# Autodesk Inventor assembly: Schlitten
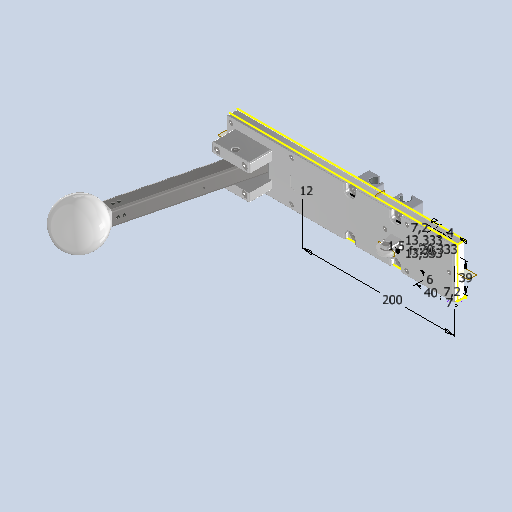
[picture p0: Inventor's stored thumbnail of the model, 512x512]
Saved by Autodesk Inventor 2025 (Build 290162010, 162A)
## iProperties
Created: 2024-11-25
Part Number: Schlitten
Document SubType Name: Assembly
Designer: Admin
Mass: 1140.3 g
Surface Area: 1828.97 cm^2
Volume: 452.563 cm^3
Density: 2.51965 g/cm^3
Author: Admin
## Documents named in this file (21)
- C:\Users\Admin\GIT\HDVKBM\CAD\Krandemonstrator\Schlitten.iam
- C:\Users\Admin\Documents\Inventor\Content Center Files\R2025\de-DE\BS 1804\BS 1804-2 - 2 x 10.ipt
- C:\Users\Admin\GIT\HDVKBM\CAD\Krandemonstrator\SchlittenS.ipt
- C:\Users\Admin\GIT\HDVKBM\CAD\Krandemonstrator\WJ200UM_01_10_1\WJ200UM_01_10_1.iam
- C:\Users\Admin\Documents\Inventor\Content Center Files\R2025\de-DE\DIN 7991(2)\DIN 7991 - M6x16.ipt
- C:\Users\Admin\GIT\HDVKBM\CAD\Krandemonstrator\SchlittenDeckel.ipt
- C:\Users\Admin\Documents\Inventor\Content Center Files\R2025\de-DE\AS 1427(03)\AS 1427 - M2 x 10(1).ipt
- C:\Users\Admin\GIT\HDVKBM\CAD\Krandemonstrator\UmlenkrolleHalterHeavy.iam
- C:\Users\Admin\GIT\HDVKBM\CAD\Krandemonstrator\Bedienhebel.iam
- C:\Users\Admin\GIT\HDVKBM\CAD\Krandemonstrator\SeilspannerDraht.ipt
- C:\Users\Admin\Documents\Inventor\Content Center Files\R2025\de-DE\DIN 7991(2)\DIN 7991 - M3x10.ipt
- C:\Users\Admin\GIT\HDVKBM\CAD\Krandemonstrator\SchlittenDeckelHinten.ipt
- C:\Users\Admin\GIT\HDVKBM\CAD\Krandemonstrator\SchlittenDeckelMitte.ipt
- C:\Users\Admin\GIT\HDVKBM\CAD\Krandemonstrator\Bremsbelag.ipt
- C:\Users\Admin\GIT\HDVKBM\CAD\Krandemonstrator\Magnet 5x3.ipt
- C:\Users\Admin\GIT\HDVKBM\CAD\Krandemonstrator\Druckfeder12.ipt
- C:\Users\Admin\Documents\Inventor\Content Center Files\R2025\de-DE\AS 1427(03)\AS 1427 - M3 x 6(1).ipt
- C:\Users\Admin\GIT\HDVKBM\CAD\Krandemonstrator\BremsePress.ipt
- C:\Users\Admin\GIT\HDVKBM\CAD\Krandemonstrator\Sliderhalterpress.ipt
- C:\Users\Admin\GIT\HDVKBM\CAD\Krandemonstrator\SchubstangeAPress.ipt
- C:\Users\Admin\GIT\HDVKBM\CAD\Krandemonstrator\SchubstangeAPressB.ipt
## Components (61 placed, 20 different names)
1. SchlittenS:1 — Passend:1, Passend:2, Passend:3, Passend:4, Starr:17, Starr:15, Starr:18, Starr:16, Drehbar:5, Drehbar:6, Drehbar:7, Drehbar:8, deckelHinten, Starr:10, Starr:11, Starr:2, Starr:3, Planar:3, Zylindrisch:9, Zylindrisch:15, Zylindrisch:16, Zylindrisch:17, Starr:21, deckelVorne, Starr:24, Starr:25, Starr:27, Starr:26, Zylindrisch:24, Planar:6, Drehbar:9, Zylindrisch:33, Zylindrisch:34, Zylindrisch:35, Zylindrisch:36, Planar:8, Zylindrisch:37, Zylindrisch:38, Zylindrisch:39
2. SchlittenDeckelMitte:1 — Starr:23, Starr:28, Starr:29
3. SchlittenDeckelHinten:1 — deckelHinten, Zylindrisch:18, Planar:4, Zylindrisch:19, Starr:23, Passend:25, Passend:26, Passend:27, Passend:28, Passend:29
4. SchlittenDeckel:1 — Zylindrisch:20, Zylindrisch:21, Zylindrisch:22, Zylindrisch:23, Planar:5, deckelVorne, Passend:21, Passend:22, Passend:23, Passend:24
5. BremsePress:1 — Drehbar:9
6. Sliderhalterpress:3 — Passend:36, Passend:37, Passend:38, Passend:39, Planar:8
7. AS 1427 - Metrisch M2 x 10:19 — Passend:36, Zylindrisch:34
8. AS 1427 - Metrisch M2 x 10:20 — Passend:37, Zylindrisch:33
9. AS 1427 - Metrisch M2 x 10:21 — Passend:38, Zylindrisch:35
10. AS 1427 - Metrisch M2 x 10:22 — Passend:39, Zylindrisch:36
11. SchubstangeAPress:1 — Verschiebbar:31, Planar:9, Starr:31
12. SchubstangeAPressB:1 — Verschiebbar:32, Starr:30, Starr:32
13. AS 1427 - Metrisch M3 x 6:2 — Starr:32
14. SeilspannerDraht:1 — Starr:21
15. DIN 7991 M3x10:6 — Zylindrisch:19
16. DIN 7991 M3x10:5 — Zylindrisch:18
17. UmlenkrolleHalterHeavy:1 [sub-assembly] — Planar:4
18. BS 1804 : Teil 2 2 x 10:4 — Drehbar:6
19. BS 1804 : Teil 2 2 x 10:1 — Drehbar:5
20. BS 1804 : Teil 2 2 x 10:2 — Drehbar:8
21. BS 1804 : Teil 2 2 x 10:3 — Drehbar:7
22. Druckfeder1:1 — Starr:30, Planar:9
23. AS 1427 - Metrisch M3 x 6:1 — Starr:31
24. AS 1427 - Metrisch M2 x 10:13 — Passend:30, Zylindrisch:38
25. AS 1427 - Metrisch M2 x 10:14 — Passend:31, Zylindrisch:39
26. AS 1427 - Metrisch M2 x 10:15 — Passend:32, Zylindrisch:24
27. AS 1427 - Metrisch M2 x 10:16 — Passend:33, Zylindrisch:37
28. Sliderhalterpress:2 — Passend:30, Passend:31, Passend:32, Passend:33, Planar:6, Verschiebbar:32
29. BS 1804 : Teil 2 2 x 10:5 — Starr:10
30. BS 1804 : Teil 2 2 x 10:6 — Starr:11
31. BS 1804 : Teil 2 2 x 10:7 — Starr:2
32. BS 1804 : Teil 2 2 x 10:8 — Starr:3
33. Sliderhalterpress:1 — Passend:13, Passend:14, Passend:15, Passend:16, Planar:3, Verschiebbar:31
34. AS 1427 - Metrisch M2 x 10:9 — Passend:13, Zylindrisch:16
35. AS 1427 - Metrisch M2 x 10:10 — Passend:14, Zylindrisch:17
36. AS 1427 - Metrisch M2 x 10:11 — Passend:15, Zylindrisch:15
37. AS 1427 - Metrisch M2 x 10:12 — Passend:16, Zylindrisch:9
38. WJ200UM_01_10_1:1 [sub-assembly] — Starr:15
39. WJ200UM_01_10_1:2 [sub-assembly] — Starr:16
40. WJ200UM_01_10_1:3 [sub-assembly] — Starr:17
41. WJ200UM_01_10_1:4 [sub-assembly] — Starr:18
42. DIN 7991 M6x16:1 — Passend:1
43. DIN 7991 M6x16:2 — Passend:2
44. DIN 7991 M6x16:3 — Passend:3
45. DIN 7991 M6x16:4 — Passend:4
46. Bremsbelag:2 — Starr:24
47. Bremsbelag:1 — Starr:25
48. Bedienhebel:1 [sub-assembly] — Zylindrisch:20, Zylindrisch:21, Zylindrisch:22, Zylindrisch:23, Planar:5
49. Magnet 5x3:1 — Starr:27
50. Magnet 5x3:2 — Starr:26
51. Magnet 5x3:3 — Starr:28
52. Magnet 5x3:4 — Starr:29
53. DIN 7991 M3x10:1 — Passend:21
54. DIN 7991 M3x10:2 — Passend:22
55. DIN 7991 M3x10:3 — Passend:23
56. DIN 7991 M3x10:4 — Passend:24
57. DIN 7991 M3x10:7 — Passend:25
58. DIN 7991 M3x10:8 — Passend:26
59. DIN 7991 M3x10:9 — Passend:27
60. DIN 7991 M3x10:10 — Passend:28
61. DIN 7991 M3x10:11 — Passend:29
## Relationships (79: Mate 27, WeldJoint 21, CylindricalJoint 18, PlanarJoint 6, RevoluteJoint 5, TranslationJoint 2)
- Passend:1 [Mate]: SchlittenS:1 ↔ DIN 7991 M6x16:1
- Passend:2 [Mate]: SchlittenS:1 ↔ DIN 7991 M6x16:2
- Passend:3 [Mate]: SchlittenS:1 ↔ DIN 7991 M6x16:3
- Passend:4 [Mate]: SchlittenS:1 ↔ DIN 7991 M6x16:4
- Starr:17 [WeldJoint]: SchlittenS:1 ↔ WJ200UM_01_10_1:3
- Starr:15 [WeldJoint]: SchlittenS:1 ↔ WJ200UM_01_10_1:1
- Starr:18 [WeldJoint]: SchlittenS:1 ↔ WJ200UM_01_10_1:4
- Starr:16 [WeldJoint]: SchlittenS:1 ↔ WJ200UM_01_10_1:2
- Drehbar:5 [RevoluteJoint]: SchlittenS:1 ↔ BS 1804 : Teil 2 2 x 10:1
- Drehbar:6 [RevoluteJoint]: SchlittenS:1 ↔ BS 1804 : Teil 2 2 x 10:4
- Drehbar:7 [RevoluteJoint]: SchlittenS:1 ↔ BS 1804 : Teil 2 2 x 10:3
- Drehbar:8 [RevoluteJoint]: SchlittenS:1 ↔ BS 1804 : Teil 2 2 x 10:2
- deckelHinten [WeldJoint]: SchlittenS:1 ↔ SchlittenDeckelHinten:1
- Starr:10 [WeldJoint]: SchlittenS:1 ↔ BS 1804 : Teil 2 2 x 10:5
- Starr:11 [WeldJoint]: SchlittenS:1 ↔ BS 1804 : Teil 2 2 x 10:6
- Starr:2 [WeldJoint]: SchlittenS:1 ↔ BS 1804 : Teil 2 2 x 10:7
- Starr:3 [WeldJoint]: SchlittenS:1 ↔ BS 1804 : Teil 2 2 x 10:8
- Passend:13 [Mate]: Sliderhalterpress:1 ↔ AS 1427 - Metrisch M2 x 10:9
- Passend:14 [Mate]: Sliderhalterpress:1 ↔ AS 1427 - Metrisch M2 x 10:10
- Passend:15 [Mate]: Sliderhalterpress:1 ↔ AS 1427 - Metrisch M2 x 10:11
- Passend:16 [Mate]: Sliderhalterpress:1 ↔ AS 1427 - Metrisch M2 x 10:12
- Planar:3: SchlittenS:1 ↔ Sliderhalterpress:1
- Zylindrisch:9 [CylindricalJoint]: SchlittenS:1 ↔ AS 1427 - Metrisch M2 x 10:12
- Zylindrisch:15 [CylindricalJoint]: SchlittenS:1 ↔ AS 1427 - Metrisch M2 x 10:11
- Zylindrisch:16 [CylindricalJoint]: SchlittenS:1 ↔ AS 1427 - Metrisch M2 x 10:9
- Zylindrisch:17 [CylindricalJoint]: SchlittenS:1 ↔ AS 1427 - Metrisch M2 x 10:10
- [Mate]: DIN 7991 M3x10:5 ↔ UmlenkrolleHalterHeavy:1
- [Mate]: DIN 7991 M3x10:6 ↔ UmlenkrolleHalterHeavy:1
- Zylindrisch:18 [CylindricalJoint]: SchlittenDeckelHinten:1 ↔ DIN 7991 M3x10:5
- Zylindrisch:19 [CylindricalJoint]: SchlittenDeckelHinten:1 ↔ DIN 7991 M3x10:6
- Planar:4: SchlittenDeckelHinten:1 ↔ UmlenkrolleHalterHeavy:1
- Zylindrisch:20 [CylindricalJoint]: SchlittenDeckel:1 ↔ Bedienhebel:1
- Zylindrisch:21 [CylindricalJoint]: SchlittenDeckel:1 ↔ Bedienhebel:1
- Zylindrisch:22 [CylindricalJoint]: SchlittenDeckel:1 ↔ Bedienhebel:1
- Zylindrisch:23 [CylindricalJoint]: SchlittenDeckel:1 ↔ Bedienhebel:1
- Planar:5: SchlittenDeckel:1 ↔ Bedienhebel:1
- Starr:21 [WeldJoint]: SchlittenS:1 ↔ SeilspannerDraht:1
- deckelVorne [WeldJoint]: SchlittenS:1 ↔ SchlittenDeckel:1
- Passend:21 [Mate]: SchlittenDeckel:1 ↔ DIN 7991 M3x10:1
- Passend:22 [Mate]: SchlittenDeckel:1 ↔ DIN 7991 M3x10:2
- Passend:23 [Mate]: SchlittenDeckel:1 ↔ DIN 7991 M3x10:3
- Passend:24 [Mate]: SchlittenDeckel:1 ↔ DIN 7991 M3x10:4
- Starr:23 [WeldJoint]: SchlittenDeckelMitte:1 ↔ SchlittenDeckelHinten:1
- Passend:25 [Mate]: SchlittenDeckelHinten:1 ↔ DIN 7991 M3x10:7
- Passend:26 [Mate]: SchlittenDeckelHinten:1 ↔ DIN 7991 M3x10:8
- Passend:27 [Mate]: SchlittenDeckelHinten:1 ↔ DIN 7991 M3x10:9
- Passend:28 [Mate]: SchlittenDeckelHinten:1 ↔ DIN 7991 M3x10:10
- Passend:29 [Mate]: SchlittenDeckelHinten:1 ↔ DIN 7991 M3x10:11
- Starr:24 [WeldJoint]: SchlittenS:1 ↔ Bremsbelag:2
- Starr:25 [WeldJoint]: SchlittenS:1 ↔ Bremsbelag:1
- Starr:27 [WeldJoint]: SchlittenS:1 ↔ Magnet 5x3:1
- Starr:26 [WeldJoint]: SchlittenS:1 ↔ Magnet 5x3:2
- Starr:28 [WeldJoint]: SchlittenDeckelMitte:1 ↔ Magnet 5x3:3
- Starr:29 [WeldJoint]: SchlittenDeckelMitte:1 ↔ Magnet 5x3:4
- Passend:30 [Mate]: AS 1427 - Metrisch M2 x 10:13 ↔ Sliderhalterpress:2
- Passend:31 [Mate]: AS 1427 - Metrisch M2 x 10:14 ↔ Sliderhalterpress:2
- Passend:32 [Mate]: AS 1427 - Metrisch M2 x 10:15 ↔ Sliderhalterpress:2
- Passend:33 [Mate]: AS 1427 - Metrisch M2 x 10:16 ↔ Sliderhalterpress:2
- Zylindrisch:24 [CylindricalJoint]: SchlittenS:1 ↔ AS 1427 - Metrisch M2 x 10:15
- Planar:6: SchlittenS:1 ↔ Sliderhalterpress:2
- Drehbar:9 [RevoluteJoint] (0.5 mm): SchlittenS:1 ↔ BremsePress:1
- Passend:36 [Mate]: Sliderhalterpress:3 ↔ AS 1427 - Metrisch M2 x 10:19
- Passend:37 [Mate]: Sliderhalterpress:3 ↔ AS 1427 - Metrisch M2 x 10:20
- Passend:38 [Mate]: Sliderhalterpress:3 ↔ AS 1427 - Metrisch M2 x 10:21
- Passend:39 [Mate]: Sliderhalterpress:3 ↔ AS 1427 - Metrisch M2 x 10:22
- Zylindrisch:33 [CylindricalJoint]: SchlittenS:1 ↔ AS 1427 - Metrisch M2 x 10:20
- Zylindrisch:34 [CylindricalJoint]: SchlittenS:1 ↔ AS 1427 - Metrisch M2 x 10:19
- Zylindrisch:35 [CylindricalJoint]: SchlittenS:1 ↔ AS 1427 - Metrisch M2 x 10:21
- Zylindrisch:36 [CylindricalJoint]: SchlittenS:1 ↔ AS 1427 - Metrisch M2 x 10:22
- Planar:8: SchlittenS:1 ↔ Sliderhalterpress:3
- Verschiebbar:31 [TranslationJoint]: SchubstangeAPress:1 ↔ Sliderhalterpress:1
- Zylindrisch:37 [CylindricalJoint]: SchlittenS:1 ↔ AS 1427 - Metrisch M2 x 10:16
- Zylindrisch:38 [CylindricalJoint]: SchlittenS:1 ↔ AS 1427 - Metrisch M2 x 10:13
- Zylindrisch:39 [CylindricalJoint]: SchlittenS:1 ↔ AS 1427 - Metrisch M2 x 10:14
- Verschiebbar:32 [TranslationJoint]: SchubstangeAPressB:1 ↔ Sliderhalterpress:2
- Starr:30 [WeldJoint]: SchubstangeAPressB:1 ↔ Druckfeder1:1
- Planar:9: SchubstangeAPress:1 ↔ Druckfeder1:1
- Starr:31 [WeldJoint]: SchubstangeAPress:1 ↔ AS 1427 - Metrisch M3 x 6:1
- Starr:32 [WeldJoint]: SchubstangeAPressB:1 ↔ AS 1427 - Metrisch M3 x 6:2
